# Autodesk Inventor assembly: final
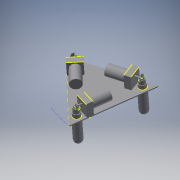
[picture p0: Inventor's stored thumbnail of the model, 180x180]
Saved by Autodesk Inventor 2018 (Build 220112000, 112)
## iProperties
Created: 2019-05-29
Part Number: final
Document SubType Name: Assembly
Designer: DELL
Author: DELL
## Documents named in this file (6)
- C:\Users\DELL\Downloads\final.iam
- C:\Users\DELL\Downloads\base1.ipt
- C:\Users\DELL\Downloads\guide1.ipt
- C:\Users\DELL\Downloads\pusher.ipt
- C:\Users\DELL\Downloads\cammotor.iam
- C:\Users\DELL\Downloads\Assembly2.iam
## Components (13 placed, 5 different names)
1. base1:1 — Rotational:1, Rotational:2, Rotational:3, Mate:6, Flush:2, Mate:8, Flush:3, Rotational:4, Rotational:5, Rotational:6, Mate:12, Flush:4
2. guide1:1 — Rotational:1, Mate:1
3. guide1:2 — Rotational:2, Mate:2
4. guide1:3 — Rotational:3, Mate:13
5. pusher:1 — Mate:1, Mate:9
6. pusher:2 — Mate:2, Mate:7
7. cammotor:1 [sub-assembly] — Mate:12, Flush:4, Mate:14
8. cammotor:2 [sub-assembly] — Mate:6, Flush:2, Mate:7
9. cammotor:3 [sub-assembly] — Mate:8, Flush:3, Mate:9
10. Assembly2:1 [sub-assembly] — Rotational:4
11. Assembly2:2 [sub-assembly] — Rotational:5
12. Assembly2:3 [sub-assembly] — Rotational:6
13. pusher:3 — Mate:13, Mate:14
## Relationships (18: Mate 9, RevoluteJoint 6, Flush 3)
- Rotational:1 [RevoluteJoint]: base1:1 ↔ guide1:1
- Rotational:2 [RevoluteJoint]: base1:1 ↔ guide1:2
- Rotational:3 [RevoluteJoint]: base1:1 ↔ guide1:3
- Mate:1: guide1:1 ↔ pusher:1
- Mate:2: guide1:2 ↔ pusher:2
- Mate:6: base1:1 ↔ cammotor:2
- Flush:2: base1:1 ↔ cammotor:2
- Mate:7: pusher:2 ↔ cammotor:2
- Mate:8: base1:1 ↔ cammotor:3
- Flush:3: base1:1 ↔ cammotor:3
- Mate:9: pusher:1 ↔ cammotor:3
- Rotational:4 [RevoluteJoint]: base1:1 ↔ Assembly2:1
- Rotational:5 [RevoluteJoint]: base1:1 ↔ Assembly2:2
- Rotational:6 [RevoluteJoint]: base1:1 ↔ Assembly2:3
- Mate:12: base1:1 ↔ cammotor:1
- Flush:4: base1:1 ↔ cammotor:1
- Mate:13: guide1:3 ↔ pusher:3
- Mate:14: cammotor:1 ↔ pusher:3
